# Autodesk Inventor assembly: Mah_Speakor
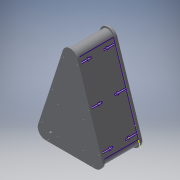
[picture p0: Inventor's stored thumbnail of the model, 180x180]
Saved by Autodesk Inventor 2016 (Build 200138000, 138)
## iProperties
Created: 2018-09-26
Part Number: Mah_Speakor
Document SubType Name: Assembly
Designer: Student
Author: Student
## Documents named in this file (7)
- C:\Users\Student\Documents\Nathan B\Mah_Speakor.iam
- C:\Users\Student\Documents\Nathan B\Nathan_Speaker.ipt
- C:\Users\Student\Documents\Nathan B\Neopixel_Stick.ipt
- C:\Users\Student\Documents\Nathan B\Eagle_Board.ipt
- C:\Users\Student\Documents\Nathan B\Nathan_LED_Speaker_Sides.ipt
- C:\Users\Student\Documents\Nathan B\Nathan_LED_Speaker_Back.ipt
- C:\Users\Student\Documents\Nathan B\Nathan_LED_Speaker_Front.ipt
## Components (8 placed, 6 different names)
1. Nathan_Speaker:1 — Mate:23, Mate:24
2. Neopixel_Stick:1 — Mate:17, Mate:18
3. Neopixel_Stick:2 — Mate:15, Mate:16
4. Neopixel_Stick:3 — Mate:19, Mate:20
5. Eagle_Board:1 — Mate:21, Mate:22
6. Nathan_LED_Speaker_Sides:1 — Mate:8, Mate:9, Mate:11, Flush:1, Mate:12, Mate:13, Flush:2, Flush:3, Mate:21
7. Nathan_LED_Speaker_Back:1 — Mate:10, Mate:11, Flush:1, Mate:13, Flush:2, Mate:14, Mate:22
8. Nathan_LED_Speaker_Front:1 — Mate:8, Mate:9, Mate:10, Mate:12, Mate:14, Flush:3, Mate:15, Mate:16, Mate:17, Mate:18, Mate:19, Mate:20, Mate:23, Mate:24
## Relationships (20: Mate 17, Flush 3)
- Mate:8: Nathan_LED_Speaker_Sides:1 ↔ Nathan_LED_Speaker_Front:1
- Mate:9: Nathan_LED_Speaker_Sides:1 ↔ Nathan_LED_Speaker_Front:1
- Mate:10 (72.136 mm): Nathan_LED_Speaker_Back:1 ↔ Nathan_LED_Speaker_Front:1
- Mate:11: Nathan_LED_Speaker_Sides:1 ↔ Nathan_LED_Speaker_Back:1
- Flush:1 (-3.175 mm): Nathan_LED_Speaker_Sides:1 ↔ Nathan_LED_Speaker_Back:1
- Mate:12: Nathan_LED_Speaker_Sides:1 ↔ Nathan_LED_Speaker_Front:1
- Mate:13: Nathan_LED_Speaker_Sides:1 ↔ Nathan_LED_Speaker_Back:1
- Flush:2 (-3.175 mm): Nathan_LED_Speaker_Sides:1 ↔ Nathan_LED_Speaker_Back:1
- Mate:14: Nathan_LED_Speaker_Back:1 ↔ Nathan_LED_Speaker_Front:1
- Flush:3 (-3.175 mm): Nathan_LED_Speaker_Sides:1 ↔ Nathan_LED_Speaker_Front:1
- Mate:15: Neopixel_Stick:2 ↔ Nathan_LED_Speaker_Front:1
- Mate:16: Neopixel_Stick:2 ↔ Nathan_LED_Speaker_Front:1
- Mate:17: Neopixel_Stick:1 ↔ Nathan_LED_Speaker_Front:1
- Mate:18: Neopixel_Stick:1 ↔ Nathan_LED_Speaker_Front:1
- Mate:19: Neopixel_Stick:3 ↔ Nathan_LED_Speaker_Front:1
- Mate:20: Neopixel_Stick:3 ↔ Nathan_LED_Speaker_Front:1
- Mate:21: Eagle_Board:1 ↔ Nathan_LED_Speaker_Sides:1
- Mate:22: Eagle_Board:1 ↔ Nathan_LED_Speaker_Back:1
- Mate:23: Nathan_Speaker:1 ↔ Nathan_LED_Speaker_Front:1
- Mate:24: Nathan_Speaker:1 ↔ Nathan_LED_Speaker_Front:1
